# Autodesk Inventor assembly: Y-Idler
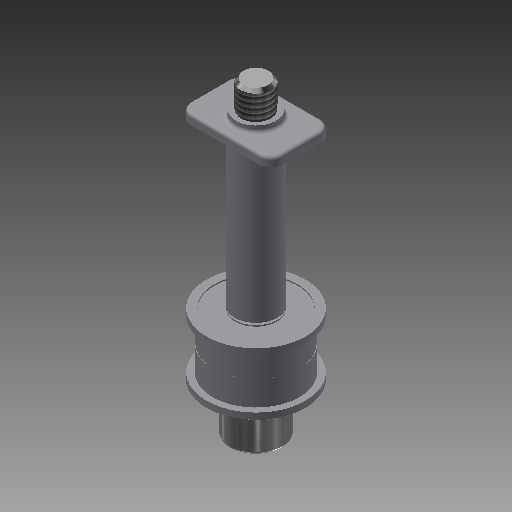
[picture p0: Inventor's stored thumbnail of the model, 512x512]
Saved by Autodesk Inventor 2018 (Build 220112000, 112)
## iProperties
Created: 2016-08-02
Part Number: Y-Idler
Document SubType Name: Assembly
Designer: User
Author: User
## Documents named in this file (6)
- C:\Users\Dan\OneDrive\SL-Inventor\The Beast v1.2 PackandGo\Workspaces\Workspace\Y-Idler.iam
- C:\Users\Dan\OneDrive\SL-Inventor\The Beast v1.2 PackandGo\Workspaces\Workspace\en-US\ANSI B18.3.1M(6)\ANSI B18.3.1M - M5x0.8 x 45(1).ipt
- C:\Users\Dan\OneDrive\SL-Inventor\The Beast v1.2 PackandGo\Workspaces\Workspace\M5 Tee Nut-Generic.ipt
- C:\Users\Dan\OneDrive\SL-Inventor\The Beast v1.2 PackandGo\Workspaces\Workspace\Flanged Bearing_CPY.ipt
- C:\Users\Dan\OneDrive\SL-Inventor\The Beast v1.2 PackandGo\Workspaces\Workspace\en-US\CSN EN 24 036\CSN EN 24 036 - M5.ipt
- C:\Users\Dan\OneDrive\SL-Inventor\The Beast v1.2 PackandGo\Workspaces\Workspace\25mmspacer.ipt
## Components (6 placed, 5 different names)
1. Forged Socket Head Cap Screw - Metric M5x0.8 x 45:1
2. M5 Tee Nut-Generic:1
3. Flanged Bearing_CPY:1
4. Flanged Bearing_CPY:2
5. CSN EN 24036 M5:1
6. 25mmspacer:1
## Relationships (7: Mate 7)
- [Mate]: Forged Socket Head Cap Screw - Metric M5x0.8 x 45:1 ↔ M5 Tee Nut-Generic:1
- [Mate]: Forged Socket Head Cap Screw - Metric M5x0.8 x 45:1 ↔ Flanged Bearing_CPY:2
- [Mate]: Forged Socket Head Cap Screw - Metric M5x0.8 x 45:1 ↔ Flanged Bearing_CPY:1
- [Mate]: Forged Socket Head Cap Screw - Metric M5x0.8 x 45:1 ↔ CSN EN 24036 M5:1
- [Mate]: Forged Socket Head Cap Screw - Metric M5x0.8 x 45:1 ↔ CSN EN 24036 M5:1
- [Mate]: Flanged Bearing_CPY:1 ↔ CSN EN 24036 M5:1
- [Mate]: Flanged Bearing_CPY:1 ↔ Flanged Bearing_CPY:2
